# Autodesk Inventor assembly: Chasis
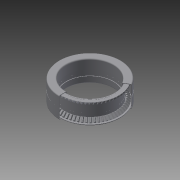
[picture p0: Inventor's stored thumbnail of the model, 180x180]
Saved by Autodesk Inventor 2015 (Build 190159000, 159)
## iProperties
Created: 2016-03-23
Part Number: Chasis
Document SubType Name: Assembly
Designer: david_000
Author: david_000
## Documents named in this file (5)
- C:\Users\david_000\Documents\Drone-Git\Drone\3D Models\Project\Chasis\Chasis.iam
- C:\Users\david_000\Documents\Drone-Git\Drone\3D Models\Project\Chasis\Top.ipt
- C:\Users\david_000\Documents\Drone-Git\Drone\3D Models\Project\Chasis\Bottom.ipt
- C:\Users\david_000\Documents\Drone-Git\Drone\3D Models\Project\Chasis\Top_Bevel.iam
- C:\Users\david_000\Documents\Drone-Git\Drone\3D Models\Project\Beveled_Ring.ipt
## Components (4 placed, 4 different names)
1. Top:1 — Insert:1, Flush:1, Insert:2
2. Bottom:1 — Insert:1, Flush:1
3. Top_Bevel:1 [sub-assembly] — Insert:2, Insert:3
4. Beveled_Ring:1 — Insert:3
## Relationships (4: Insert 3, Flush 1)
- Insert:1: Top:1 ↔ Bottom:1
- Flush:1: Top:1 ↔ Bottom:1
- Insert:2 (3.175 mm): Top:1 ↔ Top_Bevel:1
- Insert:3 (3.175 mm): Top_Bevel:1 ↔ Beveled_Ring:1
